# Autodesk Inventor assembly: N_core
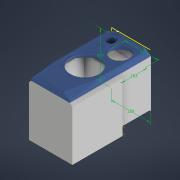
[picture p0: Inventor's stored thumbnail of the model, 180x180]
Saved by Autodesk Inventor 2022 (Build 260153070, 153G)
## iProperties
Created: 2021-11-16
Part Number: N_core
Document SubType Name: Assembly
Designer: kalugin_a
Mass: 30078.3 g
Surface Area: 26443.9 cm^2
Volume: 21974.1 cm^3
Density: 1.36881 g/cm^3
Author: kalugin_a
## Documents named in this file (15)
- C:\Users\kalugin_a\Documents\Inventor\TUTO\MELAS\Workspace\N_core.iam
- C:\Users\kalugin_a\Documents\Inventor\TUTO\MELAS\Workspace\N_Front.ipt
- C:\Users\kalugin_a\Documents\Inventor\TUTO\MELAS\Workspace\N_into_side.ipt
- C:\Users\kalugin_a\Documents\Inventor\TUTO\MELAS\Workspace\N-Back_into.ipt
- C:\Users\kalugin_a\Documents\Inventor\TUTO\MELAS\Workspace\N_Bottom.ipt
- C:\Users\kalugin_a\Documents\Inventor\TUTO\MELAS\Workspace\MID.ipt
- C:\Users\kalugin_a\Documents\Inventor\TUTO\MELAS\Workspace\N__side_sticker.ipt
- C:\Users\kalugin_a\Documents\Inventor\TUTO\MELAS\Workspace\N__side_sticker_MIR.ipt
- C:\Users\kalugin_a\Documents\Inventor\TUTO\MELAS\Workspace\WOOFER.ipt
- C:\Users\kalugin_a\Documents\Inventor\TUTO\MELAS\Workspace\MIDRange.ipt
- C:\Users\kalugin_a\Documents\Inventor\TUTO\MELAS\Workspace\Twitter.iam
- C:\Users\kalugin_a\Documents\Inventor\TUTO\MELAS\Workspace\TopCover.ipt
- C:\Users\kalugin_a\Documents\Inventor\TUTO\MELAS\Workspace\PowerSupply.ipt
- C:\Users\kalugin_a\Documents\Inventor\TUTO\MELAS\Workspace\midwall-0.ipt
- C:\Users\kalugin_a\Documents\Inventor\TUTO\MELAS\Workspace\FakeV.ipt
## Components (16 placed, 15 different names)
1. N_Front:1 — Жесткий:18
2. N_into_side:1 — Жесткий:2, Жесткий:7
3. N_into_side:2 — Жесткий:1
4. N-Back_into:1 — Жесткий:14, Жесткий:15, Жесткий:16, Жесткий:17
5. N_Flane_H — Жесткий:15
6. MID:1
7. N__side_sticker:1 — Жесткий:17
8. N__side_sticker_MIR:1 — Жесткий:14
9. N_Bottom:3 — Жесткий:1, Жесткий:2, Жесткий:16, Жесткий:18
10. TopCover:1 — Жесткий:7
11. PowerSupply:1
12. midwall-0:1 — Жесткий:12
13. FakeV:1 — Жесткий:12
14. Twitter:1 [sub-assembly]
15. MIDRange:1
16. WOOFER:2
## Relationships (9: WeldJoint 9)
- Жесткий:1 [WeldJoint]: N_into_side:2 ↔ N_Bottom:3
- Жесткий:2 [WeldJoint]: N_into_side:1 ↔ N_Bottom:3
- Жесткий:7 [WeldJoint]: N_into_side:1 ↔ TopCover:1
- Жесткий:12 [WeldJoint]: midwall-0:1 ↔ FakeV:1
- Жесткий:14 [WeldJoint]: N-Back_into:1 ↔ N__side_sticker_MIR:1
- Жесткий:15 [WeldJoint]: N-Back_into:1 ↔ N_Flane_H
- Жесткий:16 [WeldJoint]: N-Back_into:1 ↔ N_Bottom:3
- Жесткий:17 [WeldJoint]: N-Back_into:1 ↔ N__side_sticker:1
- Жесткий:18 [WeldJoint]: N_Front:1 ↔ N_Bottom:3
